# Autodesk Inventor assembly: convertor
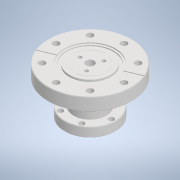
[picture p0: Inventor's stored thumbnail of the model, 180x180]
Saved by Autodesk Inventor 2020 (Build 240168000, 168)
## iProperties
Created: 2019-06-20
Part Number: convertor
Document SubType Name: Assembly
Designer: ColinP
Author: ColinP
## Documents named in this file (4)
- C:\Users\ColinP\Documents\Inventor\igor\convertor.iam
- C:\Users\ColinP\Documents\Inventor\igor\4.5 flange.ipt
- C:\Users\ColinP\Documents\Inventor\igor\FlangeCF275 Blank Modified IS.ipt
- C:\Users\ColinP\Documents\Inventor\igor\middlething.ipt
## Components (3 placed, 3 different names)
1. 4.5 flange:1 — Insert:1
2. FlangeCF275 Blank Modified IS:2 — Insert:2
3. middlething:1 — Insert:1, Insert:2
## Relationships (2: Insert 2)
- Insert:1 (-17.272 mm): 4.5 flange:1 ↔ middlething:1
- Insert:2 (-12.7 mm): FlangeCF275 Blank Modified IS:2 ↔ middlething:1
